# Autodesk Inventor assembly: Subsystem_2
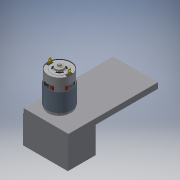
[picture p0: Inventor's stored thumbnail of the model, 180x180]
Saved by Autodesk Inventor 2019.4 (Build 234330000, 330)
## iProperties
Created: 2020-04-15
Part Number: Subsystem_2
Document SubType Name: Assembly
Designer: Niran
Author: Niran
## Documents named in this file (5)
- C:\Users\Niran\Desktop\S.Carrom_bot\Subsystem_2.iam
- C:\Users\Niran\Desktop\S.Carrom_bot\S.Part1143.ipt
- C:\Users\Niran\Desktop\S.Carrom_bot\DC Motor.ipt
- C:\Users\Niran\Desktop\S.Carrom_bot\Part13.ipt
- C:\Users\Niran\Desktop\S.Carrom_bot\Part36.ipt
## Components (5 placed, 4 different names)
1. S.Part1143:1 — Rotational:1
2. S.Part1143:2 — Rotational:1, Rotational:2, Rotational:3, Rotational:4
3. DC Motor:1 — Rotational:2
4. Part13:1 — Rotational:4
5. Part36:1 — Rotational:3
## Relationships (4: RevoluteJoint 4)
- Rotational:1 [RevoluteJoint]: S.Part1143:1 ↔ S.Part1143:2
- Rotational:2 [RevoluteJoint] (10 mm): S.Part1143:2 ↔ DC Motor:1
- Rotational:3 [RevoluteJoint] (35 mm): S.Part1143:2 ↔ Part36:1
- Rotational:4 [RevoluteJoint]: S.Part1143:2 ↔ Part13:1
